# Autodesk Inventor assembly: OmniWheel
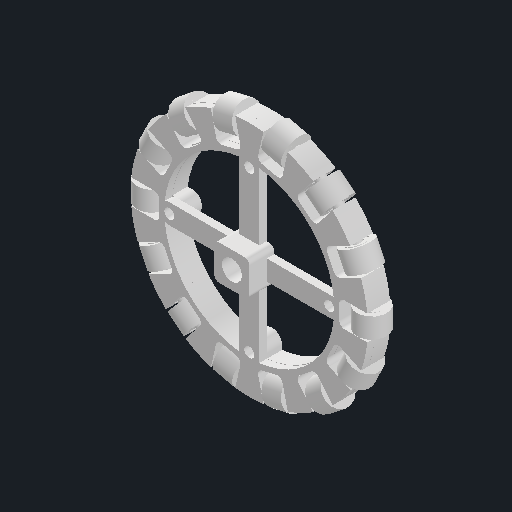
[picture p0: Inventor's stored thumbnail of the model, 512x512]
Saved by Autodesk Inventor 2024.2 (Build 282272000, 272)
## iProperties
Created: 2023-12-20
Part Number: OmniWheel
Document SubType Name: Assembly
Designer: Hanaoka
Author: Hanaoka
## Documents named in this file (4)
- G:\共有ドライブ\reRo\05_個人\hanaoka\inventor\OmniWheel.iam
- G:\共有ドライブ\reRo\05_個人\hanaoka\inventor\OmniFrame_B.ipt
- G:\共有ドライブ\reRo\05_個人\hanaoka\inventor\SideWheel.iam
- G:\共有ドライブ\reRo\05_個人\hanaoka\inventor\OmniFrame_A.ipt
## Components (16 placed, 3 different names)
1. OmniFrame_B:1 — メイト:2, メイト:3, メイト:4, メイト:5, 正接:2, 正接:3
2. OmniFrame_A:1 — フラッシュ:1, 正接:1, メイト:1, メイト:2, メイト:3, メイト:4
3. SideWheel:1 [sub-assembly] — メイト:5, 正接:2, 正接:3
4. SideWheel:2 [sub-assembly]
5. SideWheel:3 [sub-assembly]
6. SideWheel:4 [sub-assembly]
7. SideWheel:5 [sub-assembly]
8. SideWheel:6 [sub-assembly]
9. SideWheel:7 [sub-assembly]
10. SideWheel:8 [sub-assembly]
11. SideWheel:9 [sub-assembly]
12. SideWheel:10 [sub-assembly]
13. SideWheel:11 [sub-assembly]
14. SideWheel:12 [sub-assembly]
15. SideWheel:13 [sub-assembly]
16. SideWheel:14 [sub-assembly]
## Component patterns: (14 elements, first: SideWheel:1)
## Relationships (9: Mate 5, Tangent 3, Flush 1)
- フラッシュ:1 [Flush]: OmniFrame_A:1
- 正接:1 [Tangent]: OmniFrame_A:1
- メイト:1 [Mate] (6 mm): OmniFrame_A:1
- メイト:2 [Mate]: OmniFrame_B:1 ↔ OmniFrame_A:1
- メイト:3 [Mate]: OmniFrame_B:1 ↔ OmniFrame_A:1
- メイト:4 [Mate]: OmniFrame_B:1 ↔ OmniFrame_A:1
- メイト:5 [Mate] (0.5 mm): OmniFrame_B:1 ↔ SideWheel:1
- 正接:2 [Tangent] (0.025 mm): OmniFrame_B:1 ↔ SideWheel:1
- 正接:3 [Tangent] (0.025 mm): OmniFrame_B:1 ↔ SideWheel:1
